# Autodesk Inventor assembly: Assembly1
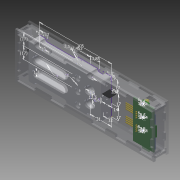
[picture p0: Inventor's stored thumbnail of the model, 180x180]
Saved by Autodesk Inventor 2015 (Build 190159000, 159)
## iProperties
Created: 2015-06-16
Part Number: Assembly1
Document SubType Name: Assembly
Designer: Openlab
Author: Openlab
## Documents named in this file (14)
- D:\Alexey\HS-Spectrophotometer\parts\Assembly1.iam
- D:\Alexey\HS-Spectrophotometer\parts\Bottom_V3.ipt
- D:\Alexey\HS-Spectrophotometer\parts\Led_Board_V1.ipt
- D:\Alexey\HS-Spectrophotometer\parts\Sensor_Board_dummy.ipt
- D:\Alexey\HS-Spectrophotometer\parts\Top_V4.ipt
- D:\Alexey\HS-Spectrophotometer\parts\Top_plate2.ipt
- D:\Alexey\HS-Spectrophotometer\parts\Large_retainer.ipt
- D:\Alexey\HS-Spectrophotometer\parts\Bottom_plate2.ipt
- D:\Alexey\HS-Spectrophotometer\parts\Left_wall.ipt
- D:\Alexey\HS-Spectrophotometer\parts\Right_wall.ipt
- D:\Alexey\HS-Spectrophotometer\parts\Cuvette_retainer2.ipt
- D:\Alexey\HS-Spectrophotometer\parts\Motherboard_assembly.iam
- D:\Alexey\HS-Spectrophotometer\parts\Back_Wall.ipt
- D:\Alexey\HS-Spectrophotometer\parts\Front_wall.ipt
## Components (14 placed, 13 different names)
1. Bottom_V3:1 — Mate:1, Mate:2, Mate:3, Mate:4, Mate:7, Mate:10, Mate:11, Mate:12, Mate:13, Mate:14, Mate:15, Mate:16, Mate:18, Mate:19, Mate:20, Mate:21, Mate:22
2. Led_Board_V1:1 — Mate:4, Mate:13, Mate:14
3. Sensor_Board_dummy:1 — Mate:7, Mate:15, Mate:16
4. Top_V4:1 — Mate:1, Mate:2, Mate:3, Mate:17
5. Top_plate2:1 — Mate:17, Mate:18, Mate:19, Mate:24, Mate:30, Mate:31, Mate:33, Mate:44, Mate:45, Mate:51
6. Large_retainer:1
7. Large_retainer:2
8. Bottom_plate2:1 — Mate:20, Mate:21, Mate:22, Mate:37, Mate:46, Mate:47, Mate:49, Mate:50
9. Left_wall:1 — Mate:24, Mate:30, Mate:35, Mate:36, Mate:44
10. Right_wall:1 — Mate:31, Mate:33, Mate:34, Mate:45
11. Cuvette_retainer2:1 — Mate:10, Mate:11, Mate:12
12. Motherboard_assembly:1 [sub-assembly] — Mate:34, Mate:35, Mate:36
13. Back_Wall:1 — Mate:37, Mate:46, Mate:47
14. Front_wall:1 — Mate:49, Mate:50, Mate:51
## Relationships (33: Mate 33)
- Mate:1: Bottom_V3:1 ↔ Top_V4:1
- Mate:2: Bottom_V3:1 ↔ Top_V4:1
- Mate:3: Bottom_V3:1 ↔ Top_V4:1
- Mate:4: Bottom_V3:1 ↔ Led_Board_V1:1
- Mate:7: Bottom_V3:1 ↔ Sensor_Board_dummy:1
- Mate:10: Bottom_V3:1 ↔ Cuvette_retainer2:1
- Mate:11: Bottom_V3:1 ↔ Cuvette_retainer2:1
- Mate:12: Bottom_V3:1 ↔ Cuvette_retainer2:1
- Mate:13: Bottom_V3:1 ↔ Led_Board_V1:1
- Mate:14: Bottom_V3:1 ↔ Led_Board_V1:1
- Mate:15: Bottom_V3:1 ↔ Sensor_Board_dummy:1
- Mate:16: Bottom_V3:1 ↔ Sensor_Board_dummy:1
- Mate:17: Top_V4:1 ↔ Top_plate2:1
- Mate:18: Bottom_V3:1 ↔ Top_plate2:1
- Mate:19: Bottom_V3:1 ↔ Top_plate2:1
- Mate:20: Bottom_V3:1 ↔ Bottom_plate2:1
- Mate:21: Bottom_V3:1 ↔ Bottom_plate2:1
- Mate:22: Bottom_V3:1 ↔ Bottom_plate2:1
- Mate:24: Top_plate2:1 ↔ Left_wall:1
- Mate:30: Top_plate2:1 ↔ Left_wall:1
- Mate:31: Top_plate2:1 ↔ Right_wall:1
- Mate:33: Top_plate2:1 ↔ Right_wall:1
- Mate:34: Right_wall:1 ↔ Motherboard_assembly:1
- Mate:35: Left_wall:1 ↔ Motherboard_assembly:1
- Mate:36: Left_wall:1 ↔ Motherboard_assembly:1
- Mate:37: Bottom_plate2:1 ↔ Back_Wall:1
- Mate:44: Top_plate2:1 ↔ Left_wall:1
- Mate:45: Top_plate2:1 ↔ Right_wall:1
- Mate:46: Bottom_plate2:1 ↔ Back_Wall:1
- Mate:47: Bottom_plate2:1 ↔ Back_Wall:1
- Mate:49: Bottom_plate2:1 ↔ Front_wall:1
- Mate:50: Bottom_plate2:1 ↔ Front_wall:1
- Mate:51: Top_plate2:1 ↔ Front_wall:1
